# Autodesk Inventor assembly: Flywheel w motor
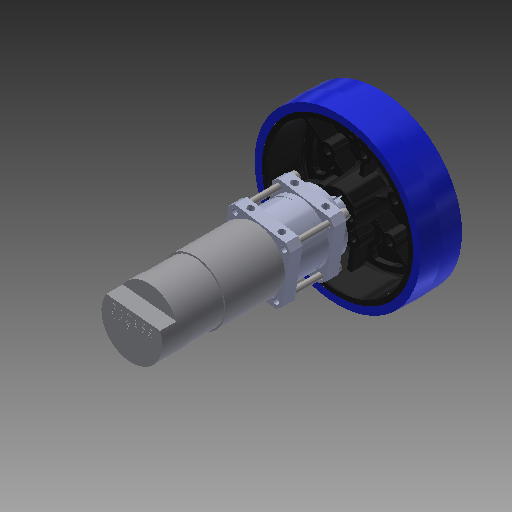
[picture p0: Inventor's stored thumbnail of the model, 512x512]
Saved by Autodesk Inventor 2017 (Build 210142000, 142)
## iProperties
Created: 2016-10-11
Part Number: Flywheel w motor
Document SubType Name: Assembly
Designer: Aditya
Author: Aditya
## Documents named in this file (4)
- C:\Users\Aditya\Documents\GitHub\RobotuxCAD\Team Robotux 15-16 Robot Cad Assets\Flywheel w motor.iam
- C:\Users\Aditya\Documents\GitHub\RobotuxCAD\Team Robotux 15-16 Robot Cad Assets\Andy Mark Parts\am-2964NeveRest-noGearbox.ipt
- C:\Users\Aditya\Documents\GitHub\RobotuxCAD\Team Robotux 15-16 Robot Cad Assets\Andy Mark Parts\am-2875+Banebots+P60+4-1.ipt
- C:\Users\Aditya\Documents\GitHub\RobotuxCAD\Team Robotux 15-16 Robot Cad Assets\Andy Mark Parts\am-2648_4inWheel8mmHubblu.ipt
## Components (3 placed, 3 different names)
1. am-2964NeveRest-noGearbox:1 — Mate:1, Mate:3
2. am-2875+Banebots+P60+4-1:1 — Mate:1, Mate:3, Mate:4, Mate:5
3. am-2648_4inWheel8mmHubblu:1 — Mate:4, Mate:5
## Relationships (4: Mate 4)
- Mate:1: am-2964NeveRest-noGearbox:1 ↔ am-2875+Banebots+P60+4-1:1
- Mate:3: am-2964NeveRest-noGearbox:1 ↔ am-2875+Banebots+P60+4-1:1
- Mate:4: am-2875+Banebots+P60+4-1:1 ↔ am-2648_4inWheel8mmHubblu:1
- Mate:5: am-2875+Banebots+P60+4-1:1 ↔ am-2648_4inWheel8mmHubblu:1
